# Autodesk Inventor assembly: End_effector_Patties
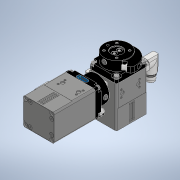
[picture p0: Inventor's stored thumbnail of the model, 180x180]
Saved by Autodesk Inventor 2021 (Build 250183000, 183)
## iProperties
Created: 2020-05-19
Part Number: End_effector_Patties
Document SubType Name: Assembly
Designer: Motius
Author: Motius
## Documents named in this file (3)
- C:\Users\avi41\Desktop\Robot Arm\CAD_files\End_effector_Patties.iam
- C:\Users\avi41\Desktop\Robot Arm\CAD_files\SCHUNK-0331220 ERD 04-40-D-H-N, 0.iam
- C:\Users\avi41\Desktop\Robot Arm\CAD_files\L_connector_actuators_endeffector.ipt
## Components (3 placed, 2 different names)
1. SCHUNK-0331220 ERD 04-40-D-H-N, 0:1 [sub-assembly] — Mate:1, Mate:2, Mate:3, Mate:4, Mate:5, Mate:6
2. SCHUNK-0331220 ERD 04-40-D-H-N, 0:2 [sub-assembly] — Mate:7, Mate:8, Mate:9
3. L_connector_actuators_endeffector:1 — Mate:4, Mate:5, Mate:6, Mate:7, Mate:8, Mate:9
## Relationships (9: Mate 9)
- Mate:1: SCHUNK-0331220 ERD 04-40-D-H-N, 0:1
- Mate:2: SCHUNK-0331220 ERD 04-40-D-H-N, 0:1
- Mate:3: SCHUNK-0331220 ERD 04-40-D-H-N, 0:1
- Mate:4: SCHUNK-0331220 ERD 04-40-D-H-N, 0:1 ↔ L_connector_actuators_endeffector:1
- Mate:5: SCHUNK-0331220 ERD 04-40-D-H-N, 0:1 ↔ L_connector_actuators_endeffector:1
- Mate:6: SCHUNK-0331220 ERD 04-40-D-H-N, 0:1 ↔ L_connector_actuators_endeffector:1
- Mate:7: SCHUNK-0331220 ERD 04-40-D-H-N, 0:2 ↔ L_connector_actuators_endeffector:1
- Mate:8: SCHUNK-0331220 ERD 04-40-D-H-N, 0:2 ↔ L_connector_actuators_endeffector:1
- Mate:9: SCHUNK-0331220 ERD 04-40-D-H-N, 0:2 ↔ L_connector_actuators_endeffector:1
